# Autodesk Inventor assembly: PCB Fixture with pin
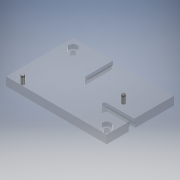
[picture p0: Inventor's stored thumbnail of the model, 180x180]
Saved by Autodesk Inventor 2017 (Build 210142000, 142)
## iProperties
Created: 2016-09-16
Part Number: PCB Fixture with pin
Document SubType Name: Assembly
Designer: Andreas Fröderberg
Author: Andreas Fröderberg
## Documents named in this file (3)
- C:\Users\Andreas Fröderberg\Documents\Inventor\PCB Fixture\PCB Fixture with pin.iam
- C:\Users\Andreas Fröderberg\Documents\Inventor\PCB Fixture\PCB FIxture 80x40.ipt
- C:\Users\Andreas Fröderberg\Documents\Inventor\PCB Fixture\CP Pin d4.ipt
## Components (3 placed, 2 different names)
1. PCB FIxture 80x40:1 — Cylindrical:1, Cylindrical:2, Flush:1, Flush:2
2. CP Pin d4:1 — Cylindrical:1, Flush:1
3. CP Pin d4:2 — Cylindrical:2, Flush:2
## Relationships (4: CylindricalJoint 2, Flush 2)
- Cylindrical:1: PCB FIxture 80x40:1 ↔ CP Pin d4:1
- Cylindrical:2: PCB FIxture 80x40:1 ↔ CP Pin d4:2
- Flush:1 (-2 mm): PCB FIxture 80x40:1 ↔ CP Pin d4:1
- Flush:2 (-2 mm): PCB FIxture 80x40:1 ↔ CP Pin d4:2
